# Autodesk Inventor assembly: Thigh
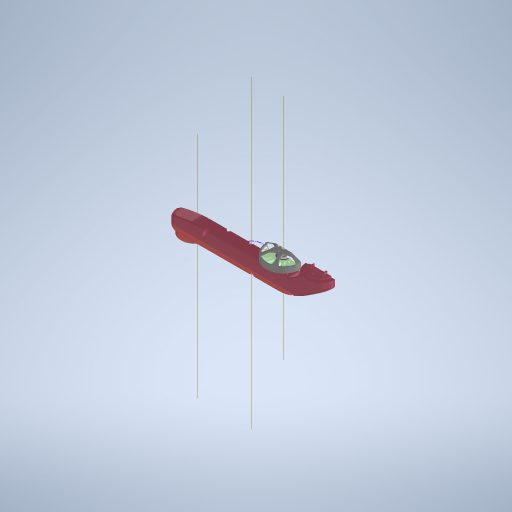
[picture p0: Inventor's stored thumbnail of the model, 512x512]
Saved by Autodesk Inventor 2023 (Build 270158000, 158)
## iProperties
Created: 2022-01-01
Part Number: Thigh
Document SubType Name: Assembly
Designer: Jochen
Author: Jochen
## Documents named in this file (10)
- D:\Projects\Lisbeth\CAD\Thigh\Thigh.iam
- D:\Projects\Lisbeth\CAD\Thigh\ThighBody.ipt
- D:\Projects\Lisbeth\CAD\Common\Encoder\encoder.iam
- D:\Projects\Lisbeth\CAD\Common\Motor\MotorModule.iam
- D:\Projects\Lisbeth\CAD\Common\Transmission\Transmission Pulley.iam
- D:\Projects\Lisbeth\CAD\Thigh\Thigh\Design Accelerator\Synchronous Belts Transmission1.iam
- D:\Projects\Lisbeth\CAD\Common\Belt Tensioner\BeltTensioner 10mm.iam
- D:\Projects\Lisbeth\CAD\Common\Belt Tensioner\MotorBeltTensioner 10mm.iam
- D:\Projects\Lisbeth\CAD\Common\Transmission\TransmissionPulleyCenter.iam
- D:\Projects\Lisbeth\CAD\Thigh\Thigh\Design Accelerator\Synchronous Belts Transmission2.iam
## Components (9 placed, 8 different names)
1. ThighBody:1 — Mate:1, Mate:2, Mate:3, Mate:4, Mate:5, Angle:1, Mate:6, Mate:14, Mate:15, Mate:23, Mate:31, Mate:32, Mate:33, Mate:34, Mate:36, Mate:37, Mate:38
2. Encoder:1 [sub-assembly] — Mate:3, Mate:5, Angle:1
3. MotorModule:1 [sub-assembly] — Mate:6, Mate:14, Mate:38
4. Transmission Pulley:1 [sub-assembly] — Mate:15, Mate:33
5. Synchronous Belts Transmission:1 [sub-assembly]
6. Belt tensioner:2 [sub-assembly] — Mate:23, Mate:34
7. MotorBeltTensioner:1 [sub-assembly] — Mate:36, Mate:37
8. TransmissionPuleyCenter:1 [sub-assembly] — Mate:31, Mate:32
9. Synchronous Belts Transmission:2 [sub-assembly]
## Relationships (17: Mate 16, Angle 1)
- Mate:1: ThighBody:1
- Mate:2: ThighBody:1
- Mate:3: ThighBody:1 ↔ Encoder:1
- Mate:4: ThighBody:1
- Mate:5: ThighBody:1 ↔ Encoder:1
- Angle:1 (0 deg): ThighBody:1 ↔ Encoder:1
- Mate:6: ThighBody:1 ↔ MotorModule:1
- Mate:14: ThighBody:1 ↔ MotorModule:1
- Mate:15: ThighBody:1 ↔ Transmission Pulley:1
- Mate:23: ThighBody:1 ↔ Belt tensioner:2
- Mate:31: ThighBody:1 ↔ TransmissionPuleyCenter:1
- Mate:32: ThighBody:1 ↔ TransmissionPuleyCenter:1
- Mate:33: ThighBody:1 ↔ Transmission Pulley:1
- Mate:34: ThighBody:1 ↔ Belt tensioner:2
- Mate:36: ThighBody:1 ↔ MotorBeltTensioner:1
- Mate:37: ThighBody:1 ↔ MotorBeltTensioner:1
- Mate:38: ThighBody:1 ↔ MotorModule:1
